# Autodesk Inventor assembly: EL2-C-100
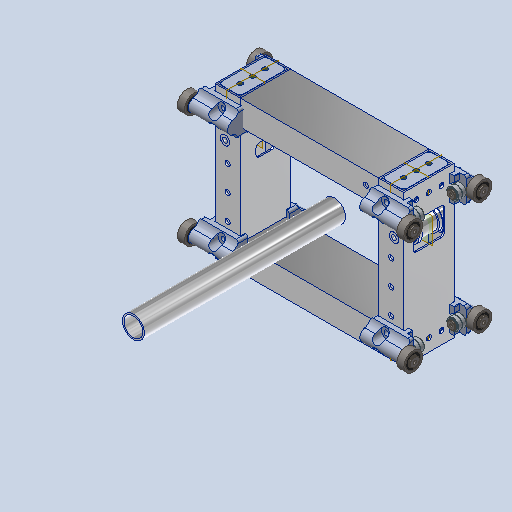
[picture p0: Inventor's stored thumbnail of the model, 512x512]
Saved by Autodesk Inventor 2023.4 (Build 274418000, 418)
## iProperties
Created: 2025-01-11
Part Number: EL2-C-100
Document SubType Name: Assembly
Designer: brand
Author: brand
## Documents named in this file (7)
- C:\Users\mavericks\Documents\GitHub\2025-ReefScape---CAD\Elevator\EL2\EL2-C-100.iam
- C:\Users\mavericks\Documents\GitHub\2025-ReefScape---CAD\Elevator\EL2\EL2-C-001.ipt
- C:\Users\mavericks\Documents\GitHub\2025-ReefScape---CAD\Elevator\EL2\EL2-005.ipt
- C:\Users\mavericks\Documents\GitHub\2025-ReefScape---CAD\Elevator\EL2\EL2-C-004.ipt
- C:\Users\mavericks\Documents\GitHub\2025-ReefScape---CAD\Elevator\EL2\EL2-C-005.ipt
- C:\Users\mavericks\Documents\GitHub\2025-ReefScape---CAD\COMMON PARTS\WCP Elevator parts\WCP-0323\WCP-0323.iam
- C:\Users\mavericks\Documents\GitHub\2025-ReefScape---CAD\Elevator\EL2\EL2-400.iam
## Components (19 placed, 6 different names)
1. EL2-C-001:1 — Flush:4, Flush:8, Mate:10, Flush:9, Flush:11
2. EL2-C-005:2 — Insert:1, Angle:1, Insert:2, Angle:2, Flush:4, Mate:10, Insert:15, Insert:16, Insert:18, Insert:21, Insert:22, Insert:25, Insert:26, Insert:27, Insert:30, Mate:11
3. EL2-C-005:1 — Insert:8, Insert:10, Insert:31, Insert:32, Insert:33, Mate:12, Flush:12, Insert:34, Insert:35, Insert:36, Insert:37, Insert:38, Insert:39, Insert:40, Insert:41
4. EL2-C-001:4 — Flush:10, Flush:11, Mate:11, Mate:12, Flush:12
5. EL2-005:1 — Insert:2, Angle:2, Flush:9
6. EL2-005:2 — Insert:8, Flush:8
7. EL2-005:3 — Insert:10, Flush:10, Insert:32, Insert:33
8. EL2-005:4 — Insert:1, Angle:1
9. EL2-C-004:1
10. WCP-0323:1 [sub-assembly] — Insert:34, Insert:35
11. WCP-0323:2 [sub-assembly] — Insert:40, Insert:41
12. WCP-0323:3 [sub-assembly] — Insert:38, Insert:39
13. WCP-0323:4 [sub-assembly] — Insert:25, Insert:27
14. WCP-0323:5 [sub-assembly] — Insert:18, Insert:26
15. WCP-0323:6 [sub-assembly] — Insert:15, Insert:16
16. WCP-0323:7 [sub-assembly] — Insert:21, Insert:22
17. WCP-0323:8 [sub-assembly] — Insert:36, Insert:37
18. EL2-400:1 [sub-assembly] — Insert:30
19. EL2-400:2 [sub-assembly] — Insert:31
## Relationships (35: Insert 24, Flush 6, Mate 3, Angle 2)
- Insert:1: EL2-C-005:2 ↔ EL2-005:4
- Angle:1 (0 deg): EL2-C-005:2 ↔ EL2-005:4
- Insert:2: EL2-C-005:2 ↔ EL2-005:1
- Angle:2 (0 deg): EL2-C-005:2 ↔ EL2-005:1
- Insert:8: EL2-C-005:1 ↔ EL2-005:2
- Insert:10: EL2-C-005:1 ↔ EL2-005:3
- Flush:4: EL2-C-001:1 ↔ EL2-C-005:2
- Flush:8: EL2-C-001:1 ↔ EL2-005:2
- Mate:10: EL2-C-001:1 ↔ EL2-C-005:2
- Flush:9: EL2-C-001:1 ↔ EL2-005:1
- Flush:10: EL2-C-001:4 ↔ EL2-005:3
- Flush:11: EL2-C-001:1 ↔ EL2-C-001:4
- Insert:15: EL2-C-005:2 ↔ WCP-0323:6
- Insert:16: EL2-C-005:2 ↔ WCP-0323:6
- Insert:18: EL2-C-005:2 ↔ WCP-0323:5
- Insert:21: EL2-C-005:2 ↔ WCP-0323:7
- Insert:22: EL2-C-005:2 ↔ WCP-0323:7
- Insert:25: EL2-C-005:2 ↔ WCP-0323:4
- Insert:26: EL2-C-005:2 ↔ WCP-0323:5
- Insert:27: EL2-C-005:2 ↔ WCP-0323:4
- Insert:30: EL2-C-005:2 ↔ EL2-400:1
- Insert:31: EL2-C-005:1 ↔ EL2-400:2
- Insert:32: EL2-C-005:1 ↔ EL2-005:3
- Insert:33: EL2-C-005:1 ↔ EL2-005:3
- Mate:11: EL2-C-005:2 ↔ EL2-C-001:4
- Mate:12: EL2-C-005:1 ↔ EL2-C-001:4
- Flush:12: EL2-C-005:1 ↔ EL2-C-001:4
- Insert:34: EL2-C-005:1 ↔ WCP-0323:1
- Insert:35: EL2-C-005:1 ↔ WCP-0323:1
- Insert:36: EL2-C-005:1 ↔ WCP-0323:8
- Insert:37: EL2-C-005:1 ↔ WCP-0323:8
- Insert:38: EL2-C-005:1 ↔ WCP-0323:3
- Insert:39: EL2-C-005:1 ↔ WCP-0323:3
- Insert:40: EL2-C-005:1 ↔ WCP-0323:2
- Insert:41: EL2-C-005:1 ↔ WCP-0323:2
